# Autodesk Inventor assembly: 옆판베어링결합_왼쪽
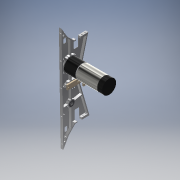
[picture p0: Inventor's stored thumbnail of the model, 180x180]
Saved by Autodesk Inventor 2017 (Build 210142000, 142)
## iProperties
Part Number: 옆판베어링결합_왼쪽
Material: 일반
Document SubType Name: Assembly
Designer: minom
Mass: 657.63 g
Surface Area: 672 cm^2
Volume: 211.202 cm^3
Density: 3.11374 g/cm^3
Author: minom
## Documents named in this file (5)
- C:\Users\minom\Documents\Inventor\Projects\2017 IRC Sumo Mino ver.2\옆판베어링결합_왼쪽.iam
- C:\Users\minom\Documents\Inventor\Projects\2017 IRC Sumo Mino ver.2\옆판_왼쪽.ipt
- C:\Users\minom\Documents\Inventor\Projects\2017 IRC Sumo Mino ver.2\FL6700ZZ.ipt
- C:\Users\minom\Documents\Inventor\Projects\2017 IRC Sumo Mino ver.2\IG-42GM_motor.ipt
- C:\Users\minom\Documents\Inventor\Projects\2017 IRC Sumo Mino ver.2\옆면PSD받침대.ipt
## Components (5 placed, 4 different names)
1. 옆판_왼쪽:1 — 메이트:1, 메이트:2, 메이트:3, 메이트:4, 메이트:5, 메이트:6, 메이트:7, 메이트:8, 메이트:9
2. FL6700ZZ:1 — 메이트:2, 메이트:3
3. FL6700ZZ:2 — 메이트:1, 메이트:4
4. IG-42GM_motor:1 — 메이트:5, 메이트:6
5. 옆면PSD받침대:1 — 메이트:7, 메이트:8, 메이트:9
## Relationships (9: Mate 9)
- 메이트:1 [Mate]: 옆판_왼쪽:1 ↔ FL6700ZZ:2
- 메이트:2 [Mate]: 옆판_왼쪽:1 ↔ FL6700ZZ:1
- 메이트:3 [Mate]: 옆판_왼쪽:1 ↔ FL6700ZZ:1
- 메이트:4 [Mate]: 옆판_왼쪽:1 ↔ FL6700ZZ:2
- 메이트:5 [Mate]: 옆판_왼쪽:1 ↔ IG-42GM_motor:1
- 메이트:6 [Mate]: 옆판_왼쪽:1 ↔ IG-42GM_motor:1
- 메이트:7 [Mate]: 옆판_왼쪽:1 ↔ 옆면PSD받침대:1
- 메이트:8 [Mate]: 옆판_왼쪽:1 ↔ 옆면PSD받침대:1
- 메이트:9 [Mate]: 옆판_왼쪽:1 ↔ 옆면PSD받침대:1
